# Autodesk Inventor assembly: Camera With Lens 1764
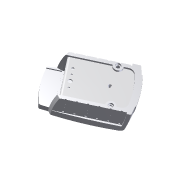
[picture p0: Inventor's stored thumbnail of the model, 180x180]
Saved by Autodesk Inventor 2011 (Build 150239000, 239)
## iProperties
Created: 2009-02-22
Part Number: Camera With Lens 1764
Document SubType Name: Assembly
Designer: jedgar
Author: jedgar
## Documents named in this file (3)
- R:\2010-2011\CMO\Web Site\CADalog\Electonics\Camera 1764\Camera With Lens 1764.iam
- R:\2010-2011\CMO\Web Site\CADalog\Electonics\Camera 1764\Camera Lens 1764.ipt
- R:\2010-2011\CMO\Web Site\CADalog\Electonics\Camera 1764\Camera 1764.ipt
## Components (2 placed, 2 different names)
1. Camera Lens 1764:1 — Mate:1, Mate:2, Mate:3, Mate:4, Mate:7
2. Camera 1764:1 — Mate:5, Mate:7, Angle:1
## Relationships (8: Mate 7, Angle 1)
- Mate:1: Camera Lens 1764:1
- Mate:2: Camera Lens 1764:1
- Mate:3: Camera Lens 1764:1
- Mate:4: Camera Lens 1764:1
- Mate:5: Camera 1764:1
- Mate:6
- Mate:7: Camera Lens 1764:1 ↔ Camera 1764:1
- Angle:1 (90 deg): Camera 1764:1
